# Autodesk Inventor assembly: Ensamble_Transmision_Potencia
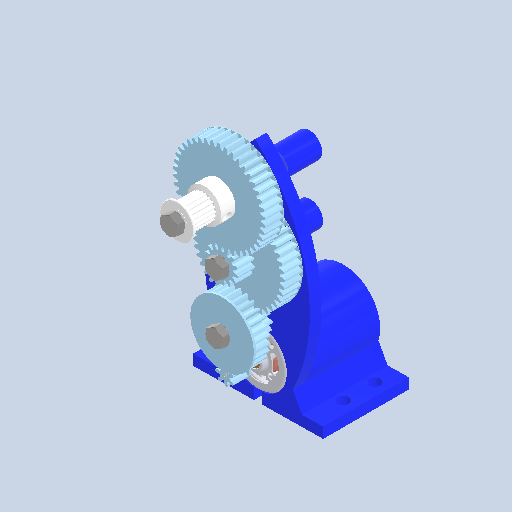
[picture p0: Inventor's stored thumbnail of the model, 512x512]
Saved by Autodesk Inventor 2022 (Build 260153000, 153)
## iProperties
Created: 2022-03-06
Part Number: Ensamble_Transmision_Potencia
Document SubType Name: Assembly
Designer: hurta
Author: hurta
## Documents named in this file (10)
- C:\Users\hurta\Documents\Universidad\NovenoSemestre\MiniProyecto1\MiniProyecto1\Diseno_Mecanico_Inventor\Transmision_Potencia\Ensamble_Transmision_Potencia.iam
- C:\Users\hurta\Documents\Universidad\NovenoSemestre\MiniProyecto1\MiniProyecto1\Diseno_Mecanico_Inventor\Soporte_MotorDC.ipt
- C:\Users\hurta\Documents\Universidad\NovenoSemestre\MiniProyecto1\MiniProyecto1\Diseno_Mecanico_Inventor\Transmision_Potencia\TrenEngrane_SegundaEtapa.iam
- C:\Users\hurta\Documents\Universidad\NovenoSemestre\MiniProyecto1\MiniProyecto1\Diseno_Mecanico_Inventor\Transmision_Potencia\TrenEngranes_SalidaPolea.iam
- C:\Users\hurta\Documents\Universidad\NovenoSemestre\MiniProyecto1\MiniProyecto1\Diseno_Mecanico_Inventor\Transmision_Potencia\TrenEngranes14_42_Dientes_TerceraEtapa.iam
- C:\Users\hurta\Documents\Universidad\NovenoSemestre\MiniProyecto1\MiniProyecto1\Diseno_Mecanico_Inventor\libreria\en-US\AS 1111\AS 1111 - M5 x 25.ipt
- C:\Users\hurta\Documents\Universidad\NovenoSemestre\MiniProyecto1\MiniProyecto1\Diseno_Mecanico_Inventor\libreria\en-US\AS 1111\AS 1111 - M5 x 45.ipt
- C:\Users\hurta\Documents\Universidad\NovenoSemestre\MiniProyecto1\MiniProyecto1\Diseno_Mecanico_Inventor\Pieza_ajuste_etapa_engrane_final.ipt
- C:\Users\hurta\Documents\Universidad\NovenoSemestre\MiniProyecto1\MiniProyecto1\Diseno_Mecanico_Inventor\Transmision_Potencia\MotorDC\MotorDCDC Motor 12V - STEP.iam
- C:\Users\hurta\Documents\Universidad\NovenoSemestre\MiniProyecto1\MiniProyecto1\Diseno_Mecanico_Inventor\Transmision_Potencia\Engrane7Dientes.ipt
## Components (10 placed, 9 different names)
1. Soporte_MotorDC:1 — Mate:1, Mate:2, Mate:3, Mate:5, Mate:16
2. TrenEngrane_SegundaEtapa:1 [sub-assembly] — Mate:1, Mate:7, Mate:8, Mate:15, Mate:18
3. TrenEngranes_SalidaPolea:1 [sub-assembly] — Mate:3, Mate:6, Mate:11, Mate:12, Mate:14
4. TrenEngranes14_42_Dientes_TerceraEtapa:1 [sub-assembly] — Mate:2, Mate:5, Mate:6, Mate:9, Mate:10, Mate:15
5. AS 1111 - Metric M5 x 25:1 — Mate:9, Mate:10
6. AS 1111 - Metric M5 x 25:2 — Mate:7, Mate:8
7. AS 1111 - Metric M5 x 45:1 — Mate:11, Mate:12, Mate:13
8. Pieza_ajuste_etapa_engrane_final:1 — Mate:13, Mate:14
9. MotorDCDC Motor 12V - STEP:1 [sub-assembly] — Mate:16, Mate:17, Flush:1
10. Engrane7Dientes:1 — Mate:17, Flush:1, Mate:18
## Relationships (18: Mate 17, Flush 1)
- Mate:1: Soporte_MotorDC:1 ↔ TrenEngrane_SegundaEtapa:1
- Mate:2: Soporte_MotorDC:1 ↔ TrenEngranes14_42_Dientes_TerceraEtapa:1
- Mate:3: Soporte_MotorDC:1 ↔ TrenEngranes_SalidaPolea:1
- Mate:5: Soporte_MotorDC:1 ↔ TrenEngranes14_42_Dientes_TerceraEtapa:1
- Mate:6: TrenEngranes_SalidaPolea:1 ↔ TrenEngranes14_42_Dientes_TerceraEtapa:1
- Mate:7: TrenEngrane_SegundaEtapa:1 ↔ AS 1111 - Metric M5 x 25:2
- Mate:8: TrenEngrane_SegundaEtapa:1 ↔ AS 1111 - Metric M5 x 25:2
- Mate:9: TrenEngranes14_42_Dientes_TerceraEtapa:1 ↔ AS 1111 - Metric M5 x 25:1
- Mate:10: TrenEngranes14_42_Dientes_TerceraEtapa:1 ↔ AS 1111 - Metric M5 x 25:1
- Mate:11: TrenEngranes_SalidaPolea:1 ↔ AS 1111 - Metric M5 x 45:1
- Mate:12: TrenEngranes_SalidaPolea:1 ↔ AS 1111 - Metric M5 x 45:1
- Mate:13: AS 1111 - Metric M5 x 45:1 ↔ Pieza_ajuste_etapa_engrane_final:1
- Mate:14: TrenEngranes_SalidaPolea:1 ↔ Pieza_ajuste_etapa_engrane_final:1
- Mate:15: TrenEngrane_SegundaEtapa:1 ↔ TrenEngranes14_42_Dientes_TerceraEtapa:1
- Mate:16: Soporte_MotorDC:1 ↔ MotorDCDC Motor 12V - STEP:1
- Mate:17: MotorDCDC Motor 12V - STEP:1 ↔ Engrane7Dientes:1
- Flush:1: MotorDCDC Motor 12V - STEP:1 ↔ Engrane7Dientes:1
- Mate:18: TrenEngrane_SegundaEtapa:1 ↔ Engrane7Dientes:1
